# Autodesk Inventor assembly: LowerLeg
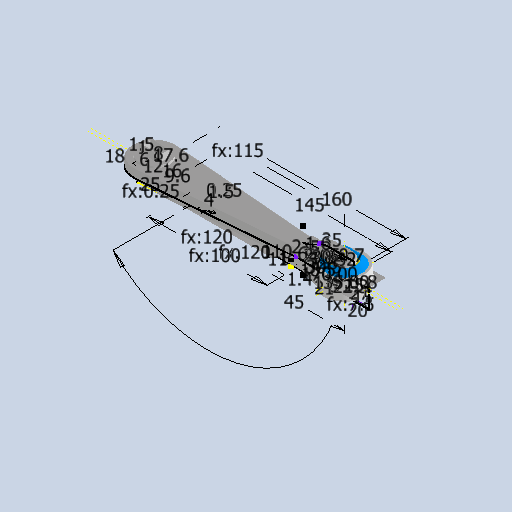
[picture p0: Inventor's stored thumbnail of the model, 512x512]
Saved by Autodesk Inventor 2023 (Build 270158000, 158)
## iProperties
Created: 2021-12-29
Part Number: LowerLeg
Document SubType Name: Assembly
Designer: Jochen
Author: Jochen
## Documents named in this file (3)
- D:\Projects\Lisbeth\CAD\LowerLeg\LowerLeg.iam
- D:\Projects\Lisbeth\CAD\LowerLeg\LowerLegBody.ipt
- D:\Projects\Lisbeth\CAD\foot\Foot.iam
## Components (2 placed, 2 different names)
1. LowerLegBody:1 — Mate:2, Mate:3, Mate:4, Mate:5
2. Foot:1 [sub-assembly] — Mate:4, Mate:5, Angle:1
## Relationships (5: Mate 4, Angle 1)
- Mate:2: LowerLegBody:1
- Mate:3: LowerLegBody:1
- Mate:4: LowerLegBody:1 ↔ Foot:1
- Mate:5: LowerLegBody:1 ↔ Foot:1
- Angle:1 (-90 deg): Foot:1
